# Autodesk Inventor assembly: Upper Static Arms
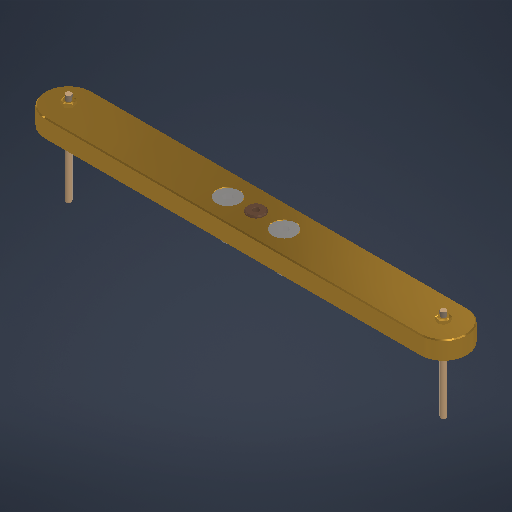
[picture p0: Inventor's stored thumbnail of the model, 512x512]
Saved by Autodesk Inventor 2027.1 (Build 311270010, 270A)
## iProperties
Created: 2025-09-16
Part Number: Upper Static Arms
Document SubType Name: Assembly
Designer: SD
Mass: 523.063 g
Surface Area: 208.84 cm^2
Volume: 61.7709 cm^3
Density: 8.46779 g/cm^3
Project: Automatic Tea Steeping mechanism
BOM-Mass: 0.52306
BOM-Area: 0.021
Author: SD
Title: Upper Static Arms
## Documents named in this file (6)
- C:\Users\Gamer\Documents\Projects\Auto Tea Steeper\Public Version\Automatic Tea Steeper\CAD\Workspace\Upper Static Arms.iam
- C:\Users\Gamer\Documents\Projects\Auto Tea Steeper\Public Version\Automatic Tea Steeper\CAD\Workspace\Brass Plate.ipt
- C:\Users\Gamer\Documents\Projects\Auto Tea Steeper\Public Version\Automatic Tea Steeper\CAD\Workspace\Domed End Rod 40mm.ipt
- C:\Users\Gamer\Documents\Projects\Auto Tea Steeper\Public Version\Automatic Tea Steeper\CAD\Workspace\Hardware\Brass M3 Hex Nut.ipt
- C:\Users\Gamer\Documents\Projects\Auto Tea Steeper\Public Version\Automatic Tea Steeper\CAD\Workspace\Hardware\CSK Allen Key 6x20mm.ipt
- C:\Users\Gamer\Documents\Projects\Auto Tea Steeper\Public Version\Automatic Tea Steeper\CAD\Workspace\FM-306-10.ipt
## Components (8 placed, 5 different names)
1. Brass Plate:1 — Mate:1, Mate:2, Flush:2, Mate:3, Mate:4, Mate:6, Mate:8, Mate:9, Flush:3, Mate:10, Flush:4
2. FM-306-10:1 — Mate:3, Mate:4
3. Domed End Rod 40mm:1 — Mate:1, Flush:1, Flush:2, Mate:7
4. Domed End Rod 40mm:2 — Mate:2, Flush:1, Mate:5
5. Brass M3 Hex Nut:1 — Mate:5, Mate:6
6. Brass M3 Hex Nut:2 — Mate:7, Mate:8
7. CSK Allen Key 6x20mm:1 — Mate:9, Flush:3
8. CSK Allen Key 6x20mm:2 — Mate:10, Flush:4
## Relationships (14: Mate 10, Flush 4)
- Mate:1: Brass Plate:1 ↔ Domed End Rod 40mm:1
- Mate:2: Brass Plate:1 ↔ Domed End Rod 40mm:2
- Flush:1: Domed End Rod 40mm:1 ↔ Domed End Rod 40mm:2
- Flush:2 (-35 mm): Brass Plate:1 ↔ Domed End Rod 40mm:1
- Mate:3: Brass Plate:1 ↔ FM-306-10:1
- Mate:4: Brass Plate:1 ↔ FM-306-10:1
- Mate:5: Domed End Rod 40mm:2 ↔ Brass M3 Hex Nut:1
- Mate:6: Brass Plate:1 ↔ Brass M3 Hex Nut:1
- Mate:7: Domed End Rod 40mm:1 ↔ Brass M3 Hex Nut:2
- Mate:8: Brass Plate:1 ↔ Brass M3 Hex Nut:2
- Mate:9: Brass Plate:1 ↔ CSK Allen Key 6x20mm:1
- Flush:3: Brass Plate:1 ↔ CSK Allen Key 6x20mm:1
- Mate:10: Brass Plate:1 ↔ CSK Allen Key 6x20mm:2
- Flush:4: Brass Plate:1 ↔ CSK Allen Key 6x20mm:2
